# Autodesk Inventor assembly: EncoderBlock
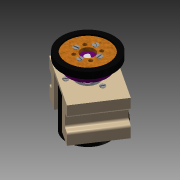
[picture p0: Inventor's stored thumbnail of the model, 180x180]
Saved by Autodesk Inventor 2014 SP1 (Build 180222100, 222)
## iProperties
Created: 2015-03-21
Part Number: EncoderBlock
Document SubType Name: Assembly
Designer: david
Mass: 144.642 g
Surface Area: 352.152 cm^2
Volume: 102.348 cm^3
Density: 1.41325 g/cm^3
EncoderBlock_BodyToWheel_Distance: 24,500 mm
EncoderBlock_InterfaceToWheel_Distance: 13,500 mm
EncoderBlock_SupportToWheel_Distance: 21,500 mm
Author: david
## Documents named in this file (7)
- C:\Users\asus\Documents\Autodesk\Projects\AUSBEEDone\Components\EncoderBlock.iam
- C:\Users\asus\Documents\Autodesk\Projects\AUSBEEDone\Components\Encoder.ipt
- C:\Users\asus\Documents\Autodesk\Projects\AUSBEEDone\Components\EncoderWheel.ipt
- C:\Users\asus\Documents\Autodesk\Projects\AUSBEEDone\Components\EncoderWheelInterface.ipt
- C:\Users\asus\Documents\Autodesk\Projects\AUSBEEDone\Components\Fasteners\Screw_CountersunkHead_3x16.ipt
- C:\Users\asus\Documents\Autodesk\Projects\AUSBEEDone\Components\EncoderSupportInside.ipt
- C:\Users\asus\Documents\Autodesk\Projects\AUSBEEDone\Components\Fasteners\Screw_CountersunkHead_3x10.ipt
## Components (12 placed, 6 different names)
1. Encoder:1 — Insert:1, Angle:1, Angle:2, Cylindrical:1, Cylindrical:2, Cylindrical:3, Mate:7, Mate:8, Mate:9, Mate:10
2. EncoderWheel:1 — Mate:1, Mate:2, Mate:4, Mate:5, Mate:6, Flush:1, Flush:2, Flush:3, Flush:4
3. EncoderWheelInterface:1 — Insert:1, Angle:1, Angle:2, Mate:1, Mate:3, Insert:2, Tangent:1, Tangent:2, Tangent:3
4. Screw_CountersunkHead_3x16:1 — Mate:5, Tangent:2, Flush:4
5. Screw_CountersunkHead_3x16:2 — Mate:2, Mate:3, Flush:1
6. Screw_CountersunkHead_3x16:4 — Insert:2
7. Screw_CountersunkHead_3x16:5 — Mate:4, Tangent:1, Flush:2
8. Screw_CountersunkHead_3x16:6 — Mate:6, Tangent:3, Flush:3
9. EncoderSupportInside:1 — Cylindrical:4, Cylindrical:5, Cylindrical:6, Mate:10
10. Screw_CountersunkHead_3x10:1 — Cylindrical:2, Mate:8, Cylindrical:5
11. Screw_CountersunkHead_3x10:2 — Cylindrical:1, Mate:7, Cylindrical:4
12. Screw_CountersunkHead_3x10:3 — Cylindrical:3, Mate:9, Cylindrical:6
## Relationships (27: Mate 10, CylindricalJoint 6, Flush 4, Tangent 3, Insert 2, Angle 2)
- Insert:1: Encoder:1 ↔ EncoderWheelInterface:1
- Angle:1 (180 deg): Encoder:1 ↔ EncoderWheelInterface:1
- Angle:2 (180 deg): Encoder:1 ↔ EncoderWheelInterface:1
- Mate:1: EncoderWheel:1 ↔ EncoderWheelInterface:1
- Mate:2: EncoderWheel:1 ↔ Screw_CountersunkHead_3x16:2
- Mate:3: EncoderWheelInterface:1 ↔ Screw_CountersunkHead_3x16:2
- Insert:2: EncoderWheelInterface:1 ↔ Screw_CountersunkHead_3x16:4
- Mate:4: EncoderWheel:1 ↔ Screw_CountersunkHead_3x16:5
- Tangent:1: EncoderWheelInterface:1 ↔ Screw_CountersunkHead_3x16:5
- Mate:5: EncoderWheel:1 ↔ Screw_CountersunkHead_3x16:1
- Tangent:2: EncoderWheelInterface:1 ↔ Screw_CountersunkHead_3x16:1
- Mate:6: EncoderWheel:1 ↔ Screw_CountersunkHead_3x16:6
- Tangent:3: EncoderWheelInterface:1 ↔ Screw_CountersunkHead_3x16:6
- Flush:1: EncoderWheel:1 ↔ Screw_CountersunkHead_3x16:2
- Flush:2: EncoderWheel:1 ↔ Screw_CountersunkHead_3x16:5
- Flush:3: EncoderWheel:1 ↔ Screw_CountersunkHead_3x16:6
- Flush:4: EncoderWheel:1 ↔ Screw_CountersunkHead_3x16:1
- Cylindrical:1: Encoder:1 ↔ Screw_CountersunkHead_3x10:2
- Cylindrical:2: Encoder:1 ↔ Screw_CountersunkHead_3x10:1
- Cylindrical:3: Encoder:1 ↔ Screw_CountersunkHead_3x10:3
- Mate:7: Encoder:1 ↔ Screw_CountersunkHead_3x10:2
- Mate:8: Encoder:1 ↔ Screw_CountersunkHead_3x10:1
- Mate:9: Encoder:1 ↔ Screw_CountersunkHead_3x10:3
- Cylindrical:4: EncoderSupportInside:1 ↔ Screw_CountersunkHead_3x10:2
- Cylindrical:5: EncoderSupportInside:1 ↔ Screw_CountersunkHead_3x10:1
- Cylindrical:6: EncoderSupportInside:1 ↔ Screw_CountersunkHead_3x10:3
- Mate:10: Encoder:1 ↔ EncoderSupportInside:1
## Named parameters: EncoderBlock_BodyToWheel_Distance = 24.5 mm, Encoder_Shaft_Length = 15 mm, EncoderWheel_Tyre_Width = 6 mm, Encoder_Bearing_Height = 5 mm, EncoderWheel_Tyre_SideWidth = 1.5 mm, EncoderBlock_InterfaceToWheel_Distance = 13.5 mm, EncoderWheelInterface_Thickness = 9 mm, EncoderBlock_SupportToWheel_Distance = 21.5 mm, EncoderSupportInside_Front_Thickness = 3 mm
